# Autodesk Inventor assembly: palp-boron-hybrid
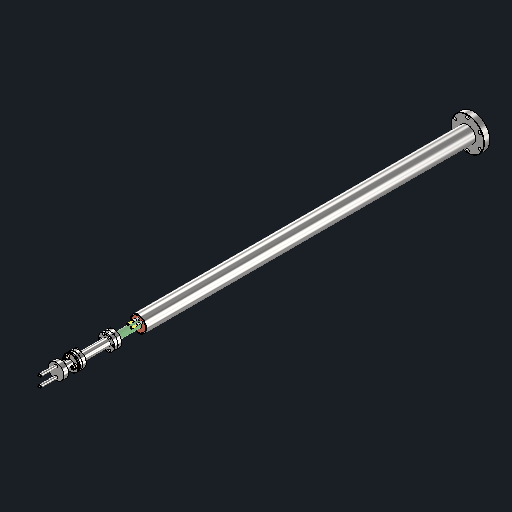
[picture p0: Inventor's stored thumbnail of the model, 512x512]
Saved by Autodesk Inventor 2026 (Build 300175050, 175E)
## iProperties
Created: 2024-05-30
Part Number: palp-boron-hybrid
Document SubType Name: Assembly
Designer: kuzmin
Author: kuzmin
## Documents named in this file (8)
- C:\Users\queez\Dropbox\Drawings\PIHTI\BoronProbe\palp-boron-hybrid.iam
- C:\Users\queez\Dropbox\Drawings\PIHTI\PALP\Prototype-PALP-ring-to-pipe-adapter_4mm.ipt
- C:\Users\queez\Dropbox\Drawings\PIHTI\ContentCenter\Ceramics\Electric-feeds\feed_4.ipt
- C:\Users\queez\Dropbox\Drawings\PIHTI\PALP\Prototype-PALP-pipe-neck-straight.ipt
- C:\Users\queez\Dropbox\Drawings\PIHTI\PALP\Prototype-PALP-CF34-flange.ipt
- C:\Users\queez\Dropbox\Drawings\PIHTI\PALP\Prototype-PALP-34pipe-with-flange.iam
- C:\Users\queez\Dropbox\Drawings\PIHTI\PALP\wire_connector.ipt
- C:\Users\queez\Dropbox\Drawings\PIHTI\BoronProbe\BoronHead.iam
## Components (9 placed, 7 different names)
1. Prototype-PALP-34pipe-with-flange:1 [sub-assembly]
2. Prototype-PALP-ring-to-pipe-adapter_4mm:1 — Rotational:6, Flush:1, Rigid:7, Rigid:8
3. feed_4:1 — Cylindrical:1, Rigid:8
4. feed_4:2 — Cylindrical:2, Rigid:7
5. Prototype-PALP-pipe-neck-straight:1 — Rotational:6, Rigid:4
6. Prototype-PALP-CF34-flange:1 — Rigid:4, Mate:5, Rigid:9
7. wire_connector:1 — Cylindrical:1
8. wire_connector:2 — Cylindrical:2
9. BoronHead:1 [sub-assembly] — Rigid:9
## Relationships (11: WeldJoint 4, Mate 2, RevoluteJoint 2, CylindricalJoint 2, Flush 1)
- [Mate]: Prototype-PALP-34pipe-with-flange:1 ↔ Prototype-PALP-ring-to-pipe-adapter_4mm:1
- [RevoluteJoint]: Prototype-PALP-34pipe-with-flange:1 ↔ Prototype-PALP-ring-to-pipe-adapter_4mm:1
- Rotational:6 [RevoluteJoint]: Prototype-PALP-ring-to-pipe-adapter_4mm:1 ↔ Prototype-PALP-pipe-neck-straight:1
- Rigid:4 [WeldJoint]: Prototype-PALP-pipe-neck-straight:1 ↔ Prototype-PALP-CF34-flange:1
- Flush:1: Prototype-PALP-ring-to-pipe-adapter_4mm:1
- Mate:5: Prototype-PALP-CF34-flange:1
- Cylindrical:1: feed_4:1 ↔ wire_connector:1
- Cylindrical:2: feed_4:2 ↔ wire_connector:2
- Rigid:7 [WeldJoint]: Prototype-PALP-ring-to-pipe-adapter_4mm:1 ↔ feed_4:2
- Rigid:8 [WeldJoint]: Prototype-PALP-ring-to-pipe-adapter_4mm:1 ↔ feed_4:1
- Rigid:9 [WeldJoint]: Prototype-PALP-CF34-flange:1 ↔ BoronHead:1
